# Autodesk Inventor assembly: High Voltage Limit Switch Standard Assembly
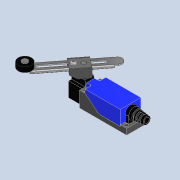
[picture p0: Inventor's stored thumbnail of the model, 180x180]
Saved by Autodesk Inventor 2022 (Build 260153000, 153)
## iProperties
Created: 2021-10-24
Part Number: High Voltage Limit Switch Standard Assembly
Document SubType Name: Assembly
Designer: Coy
Author: Coy
## Documents named in this file (4)
- H:\3D Files\Project 3D Models\Stock Parts\Sensors\Switches\High Voltage Limit Switch\High Voltage Limit Switch Standard Assembly.iam
- H:\3D Files\Project 3D Models\Stock Parts\Sensors\Switches\High Voltage Limit Switch\High Voltage Limit Switch.ipt
- H:\3D Files\Project 3D Models\Stock Parts\Sensors\Switches\High Voltage Limit Switch\High Voltage Limit Switch Arm Coupler.ipt
- H:\3D Files\Project 3D Models\Stock Parts\Sensors\Switches\High Voltage Limit Switch\High Voltage Limit Switch Arm.ipt
## Components (3 placed, 3 different names)
1. High Voltage Limit Switch:1 — Mate:1, Mate:2
2. High Voltage Limit Switch Arm Coupler:1 — Mate:1, Mate:2, Mate:3, Angle:1, Tangent:1
3. High Voltage Limit Switch Arm:1 — Mate:3, Angle:1, Tangent:1
## Relationships (5: Mate 3, Angle 1, Tangent 1)
- Mate:1: High Voltage Limit Switch:1 ↔ High Voltage Limit Switch Arm Coupler:1
- Mate:2 (1.5 mm): High Voltage Limit Switch:1 ↔ High Voltage Limit Switch Arm Coupler:1
- Mate:3: High Voltage Limit Switch Arm Coupler:1 ↔ High Voltage Limit Switch Arm:1
- Angle:1 (0 deg): High Voltage Limit Switch Arm Coupler:1 ↔ High Voltage Limit Switch Arm:1
- Tangent:1 (-6 mm): High Voltage Limit Switch Arm Coupler:1 ↔ High Voltage Limit Switch Arm:1
